# Autodesk Inventor assembly: PitchAssembly
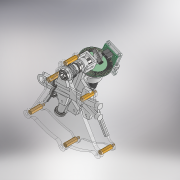
[picture p0: Inventor's stored thumbnail of the model, 180x180]
Saved by Autodesk Inventor 2018.2 (Build 222227000, 227)
## iProperties
Created: 2018-03-26
Part Number: PitchAssembly
Document SubType Name: Assembly
Designer: mansu
Author: mansu
## Documents named in this file (22)
- C:\Users\Moochster\OneDrive\Documents\2018 UBC\ELEC 391\Controller\cad\release\PitchAssembly.iam
- C:\Users\Moochster\OneDrive\Documents\2018 UBC\ELEC 391\Controller\cad\release\Rod3_8in.ipt
- C:\Users\Moochster\OneDrive\Documents\2018 UBC\ELEC 391\Controller\cad\release\ShaftArm.ipt
- C:\Users\Moochster\OneDrive\Documents\2018 UBC\ELEC 391\Controller\cad\release\R1038_ZZ_W Bearing.ipt
- C:\Users\mansu\Documents\Inventor\Content Center Files\R2018\en-US\AS 1420\AS 1420 - 1973 - M3 x 20.ipt
- C:\Users\mansu\Documents\Inventor\Content Center Files\R2018\en-US\AS 1420\AS 1420 - 1973 - M3 x 14.ipt
- C:\Users\mansu\Documents\Inventor\Content Center Files\R2018\en-US\AS 1474(1)\AS 1474 - M3(1).ipt
- C:\Users\Moochster\OneDrive\Documents\2018 UBC\ELEC 391\Controller\cad\release\RailBase.ipt
- C:\Users\Moochster\OneDrive\Documents\2018 UBC\ELEC 391\Controller\cad\release\EncoderWheelPitch.ipt
- C:\Users\Moochster\OneDrive\Documents\2018 UBC\ELEC 391\Controller\cad\release\EncoderPCBAssembly.iam
- C:\Users\Moochster\OneDrive\Documents\2018 UBC\ELEC 391\Controller\cad\release\EncoderWheelAdapterSmall.ipt
- C:\Users\Moochster\OneDrive\Documents\2018 UBC\ELEC 391\Controller\cad\release\SecondaryEncoderPCBMount.ipt
- C:\Users\Moochster\OneDrive\Documents\2018 UBC\ELEC 391\Controller\cad\release\LaserDiodeAdapter.ipt
- C:\Users\Moochster\OneDrive\Documents\2018 UBC\ELEC 391\Controller\cad\release\VLM-650-03-LPT.ipt
- C:\Users\Moochster\OneDrive\Documents\2018 UBC\ELEC 391\Controller\cad\release\GT2Shaft32T.ipt
- C:\Users\Moochster\OneDrive\Documents\2018 UBC\ELEC 391\Controller\cad\release\Fasteners\StandoffM4x20B.ipt
- C:\Users\Moochster\OneDrive\Documents\2018 UBC\ELEC 391\Controller\cad\release\RailBaseBottom.ipt
- C:\Users\Moochster\OneDrive\Documents\2018 UBC\ELEC 391\Controller\cad\release\JD5B-2655W-R.ipt
- C:\Users\Moochster\OneDrive\Documents\2018 UBC\ELEC 391\Controller\cad\release\DefaultMotorMount.ipt
- C:\Users\Moochster\OneDrive\Documents\2018 UBC\ELEC 391\Controller\cad\release\DefaultMotorMountBack.ipt
- C:\Users\Moochster\OneDrive\Documents\2018 UBC\ELEC 391\Controller\cad\release\ShaftSyncAdapter.ipt
- C:\Users\Moochster\OneDrive\Documents\2018 UBC\ELEC 391\Controller\cad\release\ForceStopper.ipt
## Components (34 placed, 21 different names)
1. Rod3_8in:1 — Mate:9, Mate:10, Mate:29, Mate:43, Mate:44, Mate:46, Flush:6, Mate:61
2. ShaftArm:1 — Mate:10, Mate:11, Flush:1, Mate:53, Mate:55, Mate:56, Mate:57, Mate:62
3. R1038_ZZ_W Bearing:1 — Mate:11, Flush:1, Tangent:3
4. AS 1420 - Metric M3 x 20:1 — Mate:27
5. AS 1420 - Metric M3 x 20:2 — Mate:21
6. AS 1420 - Metric M3 x 14:1 — Mate:23
7. AS 1420 - Metric M3 x 14:2 — Mate:25
8. AS 1474 - Metric M3:1 — Mate:21
9. AS 1474 - Metric M3:2 — Mate:23
10. AS 1474 - Metric M3:3 — Mate:25
11. AS 1474 - Metric M3:4 — Mate:27
12. RailBase:1 — Mate:29, Flush:5, Tangent:3, Insert:4, Insert:5, Insert:6, Insert:7, Insert:8, Insert:9, Mate:63, Mate:64, Mate:65, Mate:66
13. EncoderWheelPitch:1 — Mate:32, Mate:33, Mate:41, Angle:2, Mate:48, Mate:49
14. EncoderPCBAssembly:1 [sub-assembly] — Tangent:1, Tangent:2, Mate:39, Mate:45
15. EncoderWheelAdapterSmall:1 — Mate:32, Mate:33, Mate:48, Mate:50, Mate:51
16. SecondaryEncoderPCBMount:1 — Tangent:1, Tangent:2, Mate:39, Mate:45, Angle:4, Mate:58, Mate:59
17. LaserDiodeAdapter:1 — Mate:41, Mate:42, Flush:3, Angle:2, Mate:49
18. VLM-650-03-LPT:1 — Mate:42, Flush:3
19. GT2Shaft32T:1 — Mate:43
20. R1038_ZZ_W Bearing:2 — Mate:44, Flush:5
21. StandoffM4x20B:1 — Insert:7
22. StandoffM4x20B:2 — Insert:8
23. StandoffM4x20B:3 — Insert:6
24. StandoffM4x20B:4 — Insert:9
25. StandoffM4x20B:5 — Insert:5, Insert:10
26. StandoffM4x20B:6 — Insert:4
27. R1038_ZZ_W Bearing:3 — Mate:46, Mate:47
28. RailBaseBottom:1 — Mate:47, Insert:10, Angle:3, Flush:6
29. JD5B-2655W-R:1 — Mate:50, Mate:51, Mate:52, Mate:54
30. DefaultMotorMount:1 — Mate:52, Mate:53, Mate:55, Mate:56, Angle:4, Mate:58, Mate:59
31. DefaultMotorMountBack:1 — Mate:54, Mate:57
32. ShaftSyncAdapter:1 — Mate:61, Mate:62
33. ForceStopper:1 — Mate:65, Mate:66
34. ForceStopper:2 — Mate:63, Mate:64
## Relationships (53: Mate 36, Insert 7, Flush 4, Tangent 3, Angle 3)
- Mate:9: Rod3_8in:1
- Mate:10: Rod3_8in:1 ↔ ShaftArm:1
- Mate:11: ShaftArm:1 ↔ R1038_ZZ_W Bearing:1
- Flush:1 (1 mm): ShaftArm:1 ↔ R1038_ZZ_W Bearing:1
- Mate:21: AS 1420 - Metric M3 x 20:2 ↔ AS 1474 - Metric M3:1
- Mate:23: AS 1420 - Metric M3 x 14:1 ↔ AS 1474 - Metric M3:2
- Mate:25: AS 1420 - Metric M3 x 14:2 ↔ AS 1474 - Metric M3:3
- Mate:27: AS 1420 - Metric M3 x 20:1 ↔ AS 1474 - Metric M3:4
- Mate:29: Rod3_8in:1 ↔ RailBase:1
- Mate:32: EncoderWheelPitch:1 ↔ EncoderWheelAdapterSmall:1
- Mate:33 (0.1 mm): EncoderWheelPitch:1 ↔ EncoderWheelAdapterSmall:1
- Tangent:1: EncoderPCBAssembly:1 ↔ SecondaryEncoderPCBMount:1
- Tangent:2: EncoderPCBAssembly:1 ↔ SecondaryEncoderPCBMount:1
- Mate:39 (3 mm): EncoderPCBAssembly:1 ↔ SecondaryEncoderPCBMount:1
- Mate:41 (0.3 mm): EncoderWheelPitch:1 ↔ LaserDiodeAdapter:1
- Mate:42: LaserDiodeAdapter:1 ↔ VLM-650-03-LPT:1
- Flush:3 (-6 mm): LaserDiodeAdapter:1 ↔ VLM-650-03-LPT:1
- Angle:2 (0 deg): EncoderWheelPitch:1 ↔ LaserDiodeAdapter:1
- Mate:43: Rod3_8in:1 ↔ GT2Shaft32T:1
- Mate:44: Rod3_8in:1 ↔ R1038_ZZ_W Bearing:2
- Flush:5 (-0.5 mm): RailBase:1 ↔ R1038_ZZ_W Bearing:2
- Tangent:3 (0.2 mm): R1038_ZZ_W Bearing:1 ↔ RailBase:1
- Mate:45: EncoderPCBAssembly:1 ↔ SecondaryEncoderPCBMount:1
- Insert:4: RailBase:1 ↔ StandoffM4x20B:6
- Insert:5: RailBase:1 ↔ StandoffM4x20B:5
- Insert:6: RailBase:1 ↔ StandoffM4x20B:3
- Insert:7: RailBase:1 ↔ StandoffM4x20B:1
- Insert:8: RailBase:1 ↔ StandoffM4x20B:2
- Insert:9: RailBase:1 ↔ StandoffM4x20B:4
- Mate:46: Rod3_8in:1 ↔ R1038_ZZ_W Bearing:3
- Mate:47: R1038_ZZ_W Bearing:3 ↔ RailBaseBottom:1
- Insert:10: StandoffM4x20B:5 ↔ RailBaseBottom:1
- Angle:3 (0 deg): RailBaseBottom:1
- Mate:48: EncoderWheelPitch:1 ↔ EncoderWheelAdapterSmall:1
- Mate:49: EncoderWheelPitch:1 ↔ LaserDiodeAdapter:1
- Mate:50: EncoderWheelAdapterSmall:1 ↔ JD5B-2655W-R:1
- Mate:51 (1 mm): EncoderWheelAdapterSmall:1 ↔ JD5B-2655W-R:1
- Mate:52: JD5B-2655W-R:1 ↔ DefaultMotorMount:1
- Mate:53: ShaftArm:1 ↔ DefaultMotorMount:1
- Mate:54: JD5B-2655W-R:1 ↔ DefaultMotorMountBack:1
- Mate:55: ShaftArm:1 ↔ DefaultMotorMount:1
- Mate:56: ShaftArm:1 ↔ DefaultMotorMount:1
- Mate:57: ShaftArm:1 ↔ DefaultMotorMountBack:1
- Angle:4 (0 deg): SecondaryEncoderPCBMount:1 ↔ DefaultMotorMount:1
- Mate:58 (0.15 mm): SecondaryEncoderPCBMount:1 ↔ DefaultMotorMount:1
- Mate:59 (0.15 mm): SecondaryEncoderPCBMount:1 ↔ DefaultMotorMount:1
- Flush:6: Rod3_8in:1 ↔ RailBaseBottom:1
- Mate:61: Rod3_8in:1 ↔ ShaftSyncAdapter:1
- Mate:62: ShaftArm:1 ↔ ShaftSyncAdapter:1
- Mate:63: RailBase:1 ↔ ForceStopper:2
- Mate:64: RailBase:1 ↔ ForceStopper:2
- Mate:65: RailBase:1 ↔ ForceStopper:1
- Mate:66: RailBase:1 ↔ ForceStopper:1
